# Autodesk Inventor assembly: polaris_K05
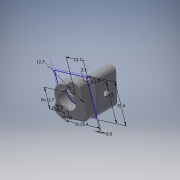
[picture p0: Inventor's stored thumbnail of the model, 180x180]
Saved by Autodesk Inventor 2016 (Build 200138000, 138)
## iProperties
Created: 2015-09-04
Part Number: polaris_K05
Document SubType Name: Assembly
Designer: HE BEC
Author: HE BEC
## Documents named in this file (4)
- C:\Users\HE BEC\Dropbox\PhD\lab\ecdl\CAD\polaris_K05.iam
- C:\Users\HE BEC\Dropbox\PhD\lab\ecdl\CAD\polaris_K05_main.ipt
- C:\Users\HE BEC\Dropbox\PhD\lab\ecdl\CAD\polaris_K05_front.ipt
- C:\Users\HE BEC\Dropbox\PhD\lab\ecdl\CAD\polaris_K05_screw.ipt
## Components (5 placed, 3 different names)
1. polaris_K05_main:1 — Mate:3, Mate:4, Mate:5, Angle:1, Angle:2, Angle:3, Flush:1, Flush:2, Flush:3
2. polaris_K05_front:1 — Tangent:2, Tangent:3
3. polaris_K05_screw:1 — Mate:5, Tangent:2, Angle:1, Flush:3
4. polaris_K05_screw:2 — Mate:4, Angle:2, Flush:2
5. polaris_K05_screw:3 — Mate:3, Angle:3, Flush:1, Tangent:3
## Relationships (11: Mate 3, Angle 3, Flush 3, Tangent 2)
- Mate:3: polaris_K05_main:1 ↔ polaris_K05_screw:3
- Mate:4: polaris_K05_main:1 ↔ polaris_K05_screw:2
- Mate:5: polaris_K05_main:1 ↔ polaris_K05_screw:1
- Tangent:2: polaris_K05_front:1 ↔ polaris_K05_screw:1
- Angle:1 (0 deg): polaris_K05_main:1 ↔ polaris_K05_screw:1
- Angle:2 (0 deg): polaris_K05_main:1 ↔ polaris_K05_screw:2
- Angle:3 (0 deg): polaris_K05_main:1 ↔ polaris_K05_screw:3
- Flush:1: polaris_K05_main:1 ↔ polaris_K05_screw:3
- Flush:2 (-0.5 mm): polaris_K05_main:1 ↔ polaris_K05_screw:2
- Tangent:3: polaris_K05_front:1 ↔ polaris_K05_screw:3
- Flush:3: polaris_K05_main:1 ↔ polaris_K05_screw:1
